# Autodesk Inventor assembly: Assembly2
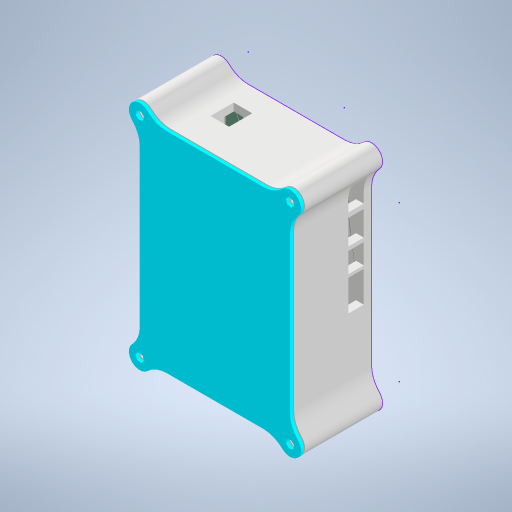
[picture p0: Inventor's stored thumbnail of the model, 512x512]
Saved by Autodesk Inventor 2024 (Build 280153000, 153)
## iProperties
Created: 2024-10-13
Part Number: Assembly2
Document SubType Name: Assembly
Designer: Lenovo
Author: Lenovo
## Documents named in this file (6)
- R:\MATERI SEMESTER 5\PRAKTIKUM IoT & JARINGAN SENSOR\SmartBuildingBox.iam
- R:\MATERI SEMESTER 5\PRAKTIKUM IoT & JARINGAN SENSOR\COVER_atas.ipt
- R:\MATERI SEMESTER 5\PRAKTIKUM IoT & JARINGAN SENSOR\TUTUP.ipt
- R:\MATERI SEMESTER 5\PRAKTIKUM IoT & JARINGAN SENSOR\Smart Building\Smart Building.iam
- R:\MATERI SEMESTER 5\PRAKTIKUM IoT & JARINGAN SENSOR\box Battery.ipt
- R:\MATERI SEMESTER 5\PRAKTIKUM IoT & JARINGAN SENSOR\Battery.ipt
## Components (6 placed, 5 different names)
1. COVER_atas:1 — Flush:1, Flush:2, Flush:3, Flush:4, Flush:5
2. TUTUP:1 — Flush:1, Flush:2
3. Smart Building:1 [sub-assembly] — Flush:3
4. box Battery:1 — Flush:4, Flush:5, Mate:1, Mate:2
5. Battery:1 — Mate:1
6. Battery:2 — Mate:2
## Relationships (7: Flush 5, Mate 2)
- Flush:1: COVER_atas:1 ↔ TUTUP:1
- Flush:2: COVER_atas:1 ↔ TUTUP:1
- Flush:3: COVER_atas:1 ↔ Smart Building:1
- Flush:4: COVER_atas:1 ↔ box Battery:1
- Flush:5: COVER_atas:1 ↔ box Battery:1
- Mate:1: box Battery:1 ↔ Battery:1
- Mate:2: box Battery:1 ↔ Battery:2
